# Autodesk Inventor assembly: Caja 2
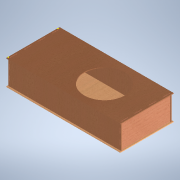
[picture p0: Inventor's stored thumbnail of the model, 180x180]
Saved by Autodesk Inventor 2020.3 (Build 243373000, 373)
## iProperties
Created: 2020-06-16
Part Number: Caja 2
Document SubType Name: Assembly
Designer: miosh
Author: miosh
## Documents named in this file (5)
- D:\Archivos Carlos\Archivos Inventor\Caja 2.iam
- D:\Archivos Carlos\Archivos Inventor\Costados pequeños.ipt
- D:\Archivos Carlos\Archivos Inventor\Frontal Secundario.ipt
- D:\Archivos Carlos\Archivos Inventor\Lado superior.ipt
- D:\Archivos Carlos\Archivos Inventor\Posterior Módulo Secundario.ipt
## Components (6 placed, 4 different names)
1. Costados pequeños:1 — Coincidencia:6, Coincidencia:9, Coincidencia:10, Nivelación:4, Coincidencia:15, Coincidencia:16
2. Costados pequeños:2 — Coincidencia:7, Coincidencia:8, Coincidencia:11, Coincidencia:12, Coincidencia:13
3. Frontal Secundario:1 — Coincidencia:6, Coincidencia:7, Coincidencia:8, Nivelación:3, Coincidencia:13, Coincidencia:14, Nivelación:5
4. Lado superior:1 — Nivelación:3, Coincidencia:9, Coincidencia:10, Coincidencia:14, Coincidencia:15, Coincidencia:17
5. Lado superior:2 — Coincidencia:11, Coincidencia:12, Nivelación:5, Nivelación:6
6. Posterior Módulo Secundario:1 — Nivelación:4, Coincidencia:16, Coincidencia:17, Nivelación:6
## Relationships (16: Mate 12, Flush 4)
- Coincidencia:6 [Mate]: Costados pequeños:1 ↔ Frontal Secundario:1
- Coincidencia:7 [Mate]: Costados pequeños:2 ↔ Frontal Secundario:1
- Coincidencia:8 [Mate]: Costados pequeños:2 ↔ Frontal Secundario:1
- Nivelación:3 [Flush]: Frontal Secundario:1 ↔ Lado superior:1
- Coincidencia:9 [Mate]: Costados pequeños:1 ↔ Lado superior:1
- Coincidencia:10 [Mate]: Costados pequeños:1 ↔ Lado superior:1
- Coincidencia:11 [Mate]: Costados pequeños:2 ↔ Lado superior:2
- Coincidencia:12 [Mate]: Costados pequeños:2 ↔ Lado superior:2
- Nivelación:4 [Flush]: Costados pequeños:1 ↔ Posterior Módulo Secundario:1
- Coincidencia:13 [Mate]: Costados pequeños:2 ↔ Frontal Secundario:1
- Coincidencia:14 [Mate]: Frontal Secundario:1 ↔ Lado superior:1
- Coincidencia:15 [Mate]: Costados pequeños:1 ↔ Lado superior:1
- Nivelación:5 [Flush]: Frontal Secundario:1 ↔ Lado superior:2
- Coincidencia:16 [Mate]: Costados pequeños:1 ↔ Posterior Módulo Secundario:1
- Coincidencia:17 [Mate]: Lado superior:1 ↔ Posterior Módulo Secundario:1
- Nivelación:6 [Flush]: Lado superior:2 ↔ Posterior Módulo Secundario:1
